# Autodesk Inventor assembly: Assembly1
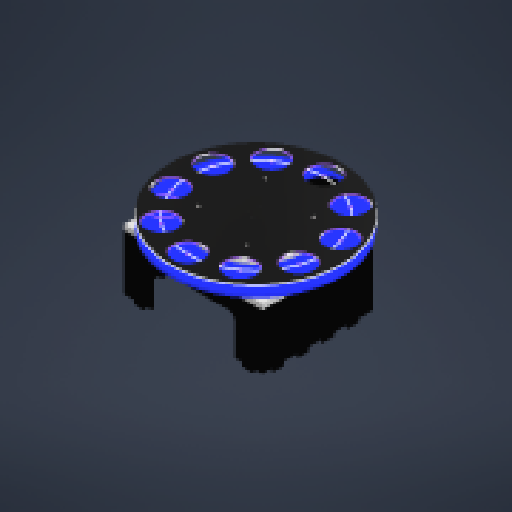
[picture p0: Inventor's stored thumbnail of the model, 512x512]
Saved by Autodesk Inventor 2027.1 (Build 311270010, 270A)
## iProperties
Created: 2026-09-28
Part Number: Assembly1
Document SubType Name: Assembly
Designer: daniel
Author: daniel
## Documents named in this file (12)
- C:\Users\danda\Documents\GitHub\MCT333_Design_of_Mechatronics_Systems_1\CAD\FEED and Sorting\Assembly1.iam
- C:\Users\danda\Documents\GitHub\MCT333_Design_of_Mechatronics_Systems_1\CAD\FEED and Sorting\Part2.ipt
- C:\Users\danda\Documents\GitHub\MCT333_Design_of_Mechatronics_Systems_1\CAD\FEED and Sorting\Part1.ipt
- C:\Users\danda\Documents\GitHub\MCT333_Design_of_Mechatronics_Systems_1\CAD\off_the_shelf_components\standard-servo-motor-black-1.snapshot.7\Assem1\Assem1.iam
- C:\Users\danda\Documents\GitHub\MCT333_Design_of_Mechatronics_Systems_1\CAD\FEED and Sorting\Part67.ipt
- C:\Users\danda\Documents\Inventor\Content Center Files\R2027\en-US\GB_T 301-1995(51000)\Rolling bearing 51109 GB_T 301-1995.ipt
- C:\Users\danda\Documents\GitHub\MCT333_Design_of_Mechatronics_Systems_1\CAD\FEED and Sorting\Part69.ipt
- C:\Users\danda\Documents\GitHub\MCT333_Design_of_Mechatronics_Systems_1\CAD\FEED and Sorting\box\MagazineBox.iam
- C:\Users\danda\Documents\Inventor\Content Center Files\R2027\en-US\ISO 7045  H\ISO 7045 - M3 x 30_ - 4.8 - H - ISO.ipt
- C:\Users\danda\Documents\Inventor\Content Center Files\R2027\en-US\ISO 7045  H\ISO 7045 - M3 x 14_ - 4.8 - H - ISO.ipt
- C:\Users\danda\Documents\Inventor\Content Center Files\R2027\en-US\ISO 4032(2)\ISO 4032 - M2.5 - ISO.ipt
- C:\Users\danda\Documents\Inventor\Content Center Files\R2027\en-US\ISO 4032(2)\ISO 4032 - M3 - ISO.ipt
## Components (24 placed, 11 different names)
1. MagazineBox:1 [sub-assembly] — Mate:2, Mate:3, Mate:4, Flush:2, Mate:9, Mate:10, Mate:11, Flush:3, Mate:18, Mate:20, Mate:22, Mate:24
2. Part2:1 — Mate:13, Mate:14, Mate:15, Mate:16, Insert:9, Insert:10, Insert:11, Insert:12
3. Part1:1 — Mate:2, Mate:3, Mate:5, Mate:6, Mate:7, Mate:8, Mate:12
4. Assem1:1 [sub-assembly] — Mate:9, Mate:10, Mate:11
5. Part67:1 — Mate:4, Flush:2, Mate:5, Flush:3
6. Rolling bearing GB/T 301-1995 Type 51000 51109:1 — Mate:12, Tangent:1, Tangent:2, Flush:4
7. Part69:1 — Tangent:2, Flush:4, Mate:13, Mate:14, Mate:15, Mate:16, Insert:5, Insert:6, Insert:7, Insert:8
8. Part69:2 — Mate:6, Mate:7, Mate:8, Tangent:1, Insert:1, Insert:2, Insert:3, Insert:4
9. ISO 7045 H M3 x 30 - 4.8 - H:1 — Insert:1, Mate:21
10. ISO 7045 H M3 x 30 - 4.8 - H:2 — Insert:2, Mate:23
11. ISO 7045 H M3 x 30 - 4.8 - H:3 — Insert:3, Mate:19
12. ISO 7045 H M3 x 30 - 4.8 - H:4 — Insert:4, Mate:17
13. ISO 7045 H M3 x 14 - 4.8 - H:1 — Insert:5
14. ISO 7045 H M3 x 14 - 4.8 - H:2 — Insert:6
15. ISO 7045 H M3 x 14 - 4.8 - H:3 — Insert:7
16. ISO 7045 H M3 x 14 - 4.8 - H:4 — Insert:8
17. ISO 4032 M2.5:1 — Insert:9
18. ISO 4032 M2.5:2 — Insert:10
19. ISO 4032 M2.5:3 — Insert:11
20. ISO 4032 M2.5:4 — Insert:12
21. ISO 4032 M3:1 — Mate:17, Mate:18
22. ISO 4032 M3:2 — Mate:19, Mate:20
23. ISO 4032 M3:3 — Mate:21, Mate:22
24. ISO 4032 M3:4 — Mate:23, Mate:24
## Relationships (40: Mate 23, Insert 12, Flush 3, Tangent 2)
- Mate:2: MagazineBox:1 ↔ Part1:1
- Mate:3: MagazineBox:1 ↔ Part1:1
- Mate:4: MagazineBox:1 ↔ Part67:1
- Flush:2: MagazineBox:1 ↔ Part67:1
- Mate:5: Part1:1 ↔ Part67:1
- Mate:6: Part1:1 ↔ Part69:2
- Mate:7: Part1:1 ↔ Part69:2
- Mate:8: Part1:1 ↔ Part69:2
- Mate:9: MagazineBox:1 ↔ Assem1:1
- Mate:10: MagazineBox:1 ↔ Assem1:1
- Mate:11: MagazineBox:1 ↔ Assem1:1
- Mate:12: Part1:1 ↔ Rolling bearing GB/T 301-1995 Type 51000 51109:1
- Tangent:1: Rolling bearing GB/T 301-1995 Type 51000 51109:1 ↔ Part69:2
- Tangent:2: Rolling bearing GB/T 301-1995 Type 51000 51109:1 ↔ Part69:1
- Flush:3: MagazineBox:1 ↔ Part67:1
- Insert:1: Part69:2 ↔ ISO 7045 H M3 x 30 - 4.8 - H:1
- Insert:2: Part69:2 ↔ ISO 7045 H M3 x 30 - 4.8 - H:2
- Insert:3: Part69:2 ↔ ISO 7045 H M3 x 30 - 4.8 - H:3
- Insert:4: Part69:2 ↔ ISO 7045 H M3 x 30 - 4.8 - H:4
- Flush:4: Rolling bearing GB/T 301-1995 Type 51000 51109:1 ↔ Part69:1
- Mate:13: Part2:1 ↔ Part69:1
- Mate:14: Part2:1 ↔ Part69:1
- Mate:15: Part2:1 ↔ Part69:1
- Mate:16: Part2:1 ↔ Part69:1
- Insert:5: Part69:1 ↔ ISO 7045 H M3 x 14 - 4.8 - H:1
- Insert:6: Part69:1 ↔ ISO 7045 H M3 x 14 - 4.8 - H:2
- Insert:7: Part69:1 ↔ ISO 7045 H M3 x 14 - 4.8 - H:3
- Insert:8: Part69:1 ↔ ISO 7045 H M3 x 14 - 4.8 - H:4
- Insert:9: Part2:1 ↔ ISO 4032 M2.5:1
- Insert:10: Part2:1 ↔ ISO 4032 M2.5:2
- Insert:11: Part2:1 ↔ ISO 4032 M2.5:3
- Insert:12: Part2:1 ↔ ISO 4032 M2.5:4
- Mate:17: ISO 7045 H M3 x 30 - 4.8 - H:4 ↔ ISO 4032 M3:1
- Mate:18: MagazineBox:1 ↔ ISO 4032 M3:1
- Mate:19: ISO 7045 H M3 x 30 - 4.8 - H:3 ↔ ISO 4032 M3:2
- Mate:20: MagazineBox:1 ↔ ISO 4032 M3:2
- Mate:21: ISO 7045 H M3 x 30 - 4.8 - H:1 ↔ ISO 4032 M3:3
- Mate:22: MagazineBox:1 ↔ ISO 4032 M3:3
- Mate:23: ISO 7045 H M3 x 30 - 4.8 - H:2 ↔ ISO 4032 M3:4
- Mate:24: MagazineBox:1 ↔ ISO 4032 M3:4
